# Autodesk Inventor assembly: WeaponAssembly
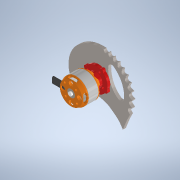
[picture p0: Inventor's stored thumbnail of the model, 180x180]
Saved by Autodesk Inventor 2020 (Build 240168000, 168)
## iProperties
Created: 2024-02-19
Part Number: WeaponAssembly
Document SubType Name: Assembly
Designer: smz3rm
Author: smz3rm
## Documents named in this file (4)
- C:\Users\smz3rm\OneDrive - BP\Documents\Battlebots\VerticalSpinner\WeaponAssembly.iam
- C:\Users\smz3rm\OneDrive - BP\Documents\Battlebots\BladeHubV1.ipt
- C:\Users\smz3rm\OneDrive - BP\Documents\Battlebots\WeaponMotorV1.ipt
- C:\Users\smz3rm\OneDrive - BP\Documents\Battlebots\WeaponV2.ipt
## Components (3 placed, 3 different names)
1. BladeHubV1:1 — Mate:1, Mate:2, Tangent:1, Mate:3, Mate:5
2. WeaponMotorV1:1 — Mate:1, Tangent:1, Mate:3
3. WeaponV2:1 — Mate:2, Mate:5
## Relationships (5: Mate 4, Tangent 1)
- Mate:1: BladeHubV1:1 ↔ WeaponMotorV1:1
- Mate:2: BladeHubV1:1 ↔ WeaponV2:1
- Tangent:1: BladeHubV1:1 ↔ WeaponMotorV1:1
- Mate:3: BladeHubV1:1 ↔ WeaponMotorV1:1
- Mate:5: BladeHubV1:1 ↔ WeaponV2:1
